# Autodesk Inventor assembly: Arm_Left
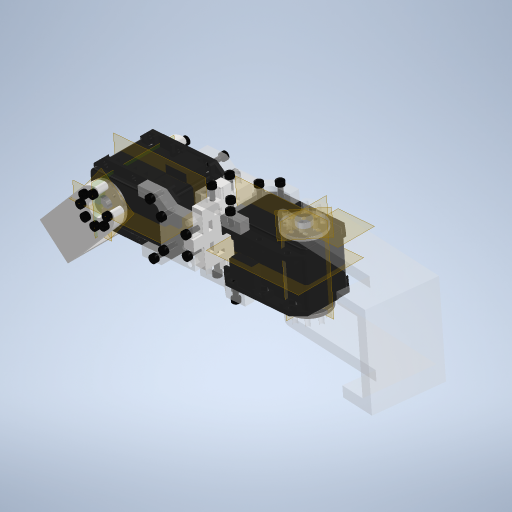
[picture p0: Inventor's stored thumbnail of the model, 512x512]
Saved by Autodesk Inventor 2024 (Build 280153000, 153)
## iProperties
Created: 2024-09-18
Part Number: Arm_Left
Document SubType Name: Assembly
Designer: Eungang
Author: Eungang
## Documents named in this file (10)
- C:\Users\Eungang\Documents\Inventor\FIGHTING_ROBOT_FINAL\부품\Arm_Left\Arm_Left.iam
- C:\Users\Eungang\Documents\Inventor\FIGHTING_ROBOT_FINAL\부품\다이나믹셀\MX-28T_R.ipt
- C:\Users\Eungang\Documents\Inventor\FIGHTING_ROBOT_FINAL\부품\아이들러\28아이들러.iam
- C:\Users\Eungang\Documents\Inventor\FIGHTING_ROBOT_FINAL\부품\혼\28Horn.ipt
- C:\Users\Eungang\Documents\Inventor\FIGHTING_ROBOT_FINAL\부품\Bolt_Washer_Nut\Arm_bolt_set_2_5_8 x 6.iam
- C:\Users\Eungang\Documents\Inventor\FIGHTING_ROBOT_FINAL\부품\Bolt_Washer_Nut\arm_motor_connect.ipt
- C:\Users\Eungang\Documents\Inventor\FIGHTING_ROBOT_FINAL\부품\Arm_Right\hand.ipt
- C:\Users\Eungang\Documents\Inventor\FIGHTING_ROBOT_FINAL\부품\Arm_Right\arm_connect_3.ipt
- C:\Users\Eungang\Documents\Inventor\FIGHTING_ROBOT_FINAL\부품\Arm_Right\arm_motor_connecter_bridge.ipt
- C:\Users\Eungang\Documents\Inventor\FIGHTING_ROBOT_FINAL\부품\Bolt_Washer_Nut\CSH-ST-M2_5-8_203.ipt
## Components (31 placed, 9 different names)
1. MX-28T_R:1 — 각도:1
2. 28아이들러:1 [sub-assembly]
3. 28Horn:1
4. Arm_bolt_set_2_5_8 x 6:1 [sub-assembly]
5. Arm_bolt_set_2_5_8 x 6:2 [sub-assembly]
6. MX-28T_R:2
7. 28아이들러:2 [sub-assembly]
8. 28Horn:2
9. Arm_bolt_set_2_5_8 x 6:3 [sub-assembly]
10. Arm_bolt_set_2_5_8 x 6:4 [sub-assembly]
11. arm_motor_connect:1
12. hand:1
13. arm_connect_3:1 — 각도:1
14. arm_motor_connecter_bridge:1
15. arm_motor_connecter_bridge:2
16. arm_motor_connecter_bridge:3
17. arm_motor_connecter_bridge:4
18. CSH-ST-M2_5-8_203:1
19. CSH-ST-M2_5-8_203:2
20. CSH-ST-M2_5-8_203:3
21. CSH-ST-M2_5-8_203:4
22. CSH-ST-M2_5-8_203:5
23. CSH-ST-M2_5-8_203:6
24. CSH-ST-M2_5-8_203:7
25. CSH-ST-M2_5-8_203:8
26. CSH-ST-M2_5-8_203:9
27. CSH-ST-M2_5-8_203:10
28. CSH-ST-M2_5-8_203:11
29. CSH-ST-M2_5-8_203:12
30. CSH-ST-M2_5-8_203:13
31. CSH-ST-M2_5-8_203:14
## Relationships (41: Insert 37, Flush 2, Mate 1, Angle 1)
- [Insert] (0.75 mm): MX-28T_R:1 ↔ 28Horn:1
- [Insert] (0.75 mm): MX-28T_R:1 ↔ 28아이들러:1
- [Insert] (0.75 mm): MX-28T_R:2 ↔ 28Horn:2
- [Insert] (0.75 mm): MX-28T_R:2 ↔ 28아이들러:2
- [Flush]: MX-28T_R:1 ↔ MX-28T_R:2
- [Flush]: MX-28T_R:1 ↔ MX-28T_R:2
- [Insert] (0.1 mm): 28Horn:2 ↔ hand:1
- [Insert]: MX-28T_R:2 ↔ arm_motor_connecter_bridge:3
- [Insert]: MX-28T_R:2 ↔ arm_motor_connecter_bridge:3
- [Insert]: MX-28T_R:2 ↔ arm_motor_connecter_bridge:4
- [Insert]: MX-28T_R:2 ↔ arm_motor_connecter_bridge:4
- [Insert]: MX-28T_R:1 ↔ arm_motor_connecter_bridge:2
- [Insert]: MX-28T_R:1 ↔ arm_motor_connecter_bridge:2
- [Insert]: MX-28T_R:1 ↔ arm_motor_connecter_bridge:1
- [Insert]: MX-28T_R:1 ↔ arm_motor_connecter_bridge:1
- [Insert]: Arm_bolt_set_2_5_8 x 6:2 ↔ arm_motor_connecter_bridge:1
- [Insert]: Arm_bolt_set_2_5_8 x 6:2 ↔ arm_motor_connecter_bridge:1
- [Mate]: arm_motor_connect:1 ↔ arm_motor_connecter_bridge:4
- [Insert] (0.1 mm): arm_motor_connect:1 ↔ arm_motor_connecter_bridge:3
- [Insert] (0.1 mm): arm_motor_connect:1 ↔ arm_motor_connecter_bridge:1
- [Insert]: Arm_bolt_set_2_5_8 x 6:4 ↔ arm_motor_connecter_bridge:3
- [Insert]: Arm_bolt_set_2_5_8 x 6:1 ↔ arm_motor_connecter_bridge:2
- [Insert]: Arm_bolt_set_2_5_8 x 6:1 ↔ arm_motor_connecter_bridge:2
- [Insert] (0.1 mm): 28Horn:1 ↔ arm_connect_3:1
- [Insert]: arm_connect_3:1 ↔ CSH-ST-M2_5-8_203:1
- [Insert]: arm_connect_3:1 ↔ CSH-ST-M2_5-8_203:2
- [Insert]: arm_connect_3:1 ↔ CSH-ST-M2_5-8_203:3
- [Insert]: arm_connect_3:1 ↔ CSH-ST-M2_5-8_203:4
- [Insert]: arm_connect_3:1 ↔ CSH-ST-M2_5-8_203:6
- [Insert]: arm_connect_3:1 ↔ CSH-ST-M2_5-8_203:5
- [Insert]: arm_connect_3:1 ↔ CSH-ST-M2_5-8_203:7
- [Insert]: arm_connect_3:1 ↔ CSH-ST-M2_5-8_203:8
- [Insert]: arm_connect_3:1 ↔ CSH-ST-M2_5-8_203:9
- [Insert]: arm_connect_3:1 ↔ CSH-ST-M2_5-8_203:10
- [Insert]: arm_connect_3:1 ↔ CSH-ST-M2_5-8_203:11
- [Insert]: arm_connect_3:1 ↔ CSH-ST-M2_5-8_203:12
- [Insert]: arm_connect_3:1 ↔ CSH-ST-M2_5-8_203:13
- [Insert]: arm_connect_3:1 ↔ CSH-ST-M2_5-8_203:14
- [Insert]: Arm_bolt_set_2_5_8 x 6:3 ↔ arm_motor_connecter_bridge:4
- [Insert]: Arm_bolt_set_2_5_8 x 6:3 ↔ arm_motor_connecter_bridge:4
- 각도:1 [Angle] (45 deg): MX-28T_R:1 ↔ arm_connect_3:1
## Named parameters: d0_d1 = 0.75 mm, d1_d2 = 0.75 mm, d29_d1 = 0.75 mm, d30_d2 = 0.75 mm, d24_d39 = 0 mm
